# Autodesk Inventor assembly: s-assy-rc_servo
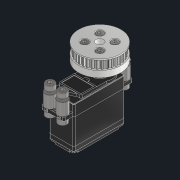
[picture p0: Inventor's stored thumbnail of the model, 180x180]
Saved by Autodesk Inventor 2022 (Build 260153000, 153)
## iProperties
Created: 2021-08-06
Part Number: s-assy-rc_servo
Document SubType Name: Assembly
Designer: yuta0
Mass: 598.977 g
Surface Area: 2161.2 cm^2
Volume: 259.929 cm^3
Density: 2.30439 g/cm^3
Author: yuta0
## Documents named in this file (8)
- C:\Users\yuta0\Documents\GitHub\catchrobo_hardware\assy-robot\s-assy-rc_servo.iam
- C:\Users\yuta0\Documents\GitHub\catchrobo_hardware\assy-robot\MG_996R.iam
- C:\Users\yuta0\Documents\GitHub\catchrobo_hardware\assy-robot\base35.ipt
- C:\Users\yuta0\Documents\GitHub\catchrobo_hardware\assy-robot\ARF-410E.ipt
- C:\Users\yuta0\Documents\GitHub\catchrobo_hardware\assy-robot\CB4-6.ipt
- C:\Users\yuta0\Documents\GitHub\catchrobo_hardware\assy-robot\CB3-12.ipt
- C:\Users\yuta0\Documents\GitHub\catchrobo_hardware\assy-robot\CB3-5.ipt
- C:\Users\yuta0\Documents\GitHub\catchrobo_hardware\assy-robot\CBSTSR4-6.ipt
## Components (19 placed, 7 different names)
1. MG_996R:1 [sub-assembly] — メイト:17, メイト:18, メイト:19, メイト:32, メイト:34, メイト:35, メイト:97, メイト:140, メイト:142, メイト:143, メイト:147
2. CB3-5:9 — メイト:96, メイト:97
3. base35:1 — メイト:17, メイト:18, メイト:19, メイト:43, メイト:44, メイト:96
4. CB3-12:1 — メイト:43, メイト:44
5. CB3-12:2
6. CB3-12:3
7. CB3-12:4
8. CB4-6:1 — メイト:34, メイト:35
9. ARF-410E:1 — メイト:32, メイト:145, メイト:146, メイト:147
10. CB4-6:10 — メイト:141, メイト:142
11. ARF-410E:2 — メイト:139, メイト:140, メイト:141, メイト:143, メイト:144
12. CB4-6:9 — メイト:139, メイト:144
13. CBSTSR4-6:6 — メイト:145, メイト:146
14. CB4-6:11
15. ARF-410E:3
16. CB4-6:12
17. ARF-410E:4
18. CB4-6:13
19. CBSTSR4-6:12
## Component patterns: (4 elements, first: CB3-12:1), (2 elements, first: CB4-6:1 + ARF-410E:1 + CB4-6:10 + ARF-410E:2 + CB4-6:9 + CBSTSR4-6:6)
## Relationships (19: Mate 19)
- メイト:17 [Mate]: MG_996R:1 ↔ base35:1
- メイト:18 [Mate]: MG_996R:1 ↔ base35:1
- メイト:19 [Mate]: MG_996R:1 ↔ base35:1
- メイト:32 [Mate]: MG_996R:1 ↔ ARF-410E:1
- メイト:34 [Mate]: MG_996R:1 ↔ CB4-6:1
- メイト:35 [Mate]: MG_996R:1 ↔ CB4-6:1
- メイト:43 [Mate]: base35:1 ↔ CB3-12:1
- メイト:44 [Mate]: base35:1 ↔ CB3-12:1
- メイト:96 [Mate]: CB3-5:9 ↔ base35:1
- メイト:97 [Mate]: MG_996R:1 ↔ CB3-5:9
- メイト:139 [Mate]: ARF-410E:2 ↔ CB4-6:9
- メイト:140 [Mate]: MG_996R:1 ↔ ARF-410E:2
- メイト:141 [Mate]: CB4-6:10 ↔ ARF-410E:2
- メイト:142 [Mate]: MG_996R:1 ↔ CB4-6:10
- メイト:143 [Mate]: MG_996R:1 ↔ ARF-410E:2
- メイト:144 [Mate] (2 mm): ARF-410E:2 ↔ CB4-6:9
- メイト:145 [Mate]: ARF-410E:1 ↔ CBSTSR4-6:6
- メイト:146 [Mate] (2 mm): ARF-410E:1 ↔ CBSTSR4-6:6
- メイト:147 [Mate]: MG_996R:1 ↔ ARF-410E:1
